# Autodesk Inventor assembly: ABD_Ankle_Version 1.0_MIR
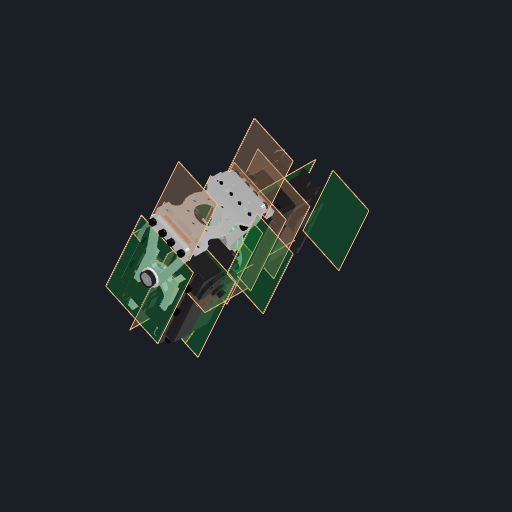
[picture p0: Inventor's stored thumbnail of the model, 512x512]
Saved by Autodesk Inventor 2024 (Build 280153000, 153)
## iProperties
Created: 2024-01-23
Part Number: ABD_Ankle_Version 1.0_MIR
Document SubType Name: Assembly
Designer: ASUS
Mass: 356.311 g
Surface Area: 603.891 cm^2
Volume: 181.117 cm^3
Author: ASUS
## Documents named in this file (21)
- C:\Users\김대겸\Desktop\2024_Robit_Hardware\ROBOCUP_2024_eindhoven\부품\Lower_Body\Anti_Backlash_Disk\ABD_Ankle_Version 1.0_MIR.iam
- C:\Users\김대겸\Desktop\2024_Robit_Hardware\ROBOCUP_2024_eindhoven\부품\ROBOTIS(Inventor 2023 ver.)\다이나믹셀\MX-106T+idle.ipt.iam
- C:\Users\김대겸\Desktop\2024_Robit_Hardware\ROBOCUP_2024_eindhoven\부품\Lower_Body\Anti_Backlash_Disk\Slider_crank_horn.ipt
- C:\Users\김대겸\Desktop\2024_Robit_Hardware\ROBOCUP_2024_eindhoven\부품\Lower_Body\Anti_Backlash_Disk\Leg_joint_slider_frame.ipt
- C:\Users\김대겸\Desktop\2024_Robit_Hardware\ROBOCUP_2024_eindhoven\부품\Lower_Body\Leg\Roll_Fixation_L.ipt
- C:\Users\김대겸\Desktop\2024_Robit_Hardware\ROBOCUP_2024_eindhoven\부품\Lower_Body\Leg\Roll_Fixation_R.ipt
- C:\Users\김대겸\Desktop\2024_Robit_Hardware\ROBOCUP_2024_eindhoven\부품\Lower_Body\Leg\Roll_Fixation_Frame.ipt
- C:\Users\김대겸\Desktop\2024_Robit_Hardware\ROBOCUP_2024_eindhoven\부품\Lower_Body\Leg\Roll_Fixation_Frame_Back.ipt
- C:\Users\김대겸\Desktop\2024_Robit_Hardware\ROBOCUP_2024_eindhoven\부품\Lower_Body\Leg\Roll_Fixation_Frameto64.ipt
- C:\Users\김대겸\Desktop\2024_Robit_Hardware\ROBOCUP_2024_eindhoven\부품\Lower_Body\Leg\106_Slider_Fixation_MIR.ipt
- C:\Users\김대겸\Desktop\2024_Robit_Hardware\ROBOCUP_2024_eindhoven\부품\Lower_Body\Hip joint of the waist\hip joint fix washer.ipt
- C:\Users\김대겸\Desktop\2024_Robit_Hardware\ROBOCUP_2024_eindhoven\부품\Lower_Body\Foot\Ankle_Footbase_Connector.ipt
- C:\Users\김대겸\Desktop\2024_Robit_Hardware\ROBOCUP_2024_eindhoven\부품\Bolt_Washer_Nut\hip_joint_fix_washer_10mm_Set.iam
- C:\Users\김대겸\Desktop\2024_Robit_Hardware\ROBOCUP_2024_eindhoven\부품\Bolt_Washer_Nut\Roll_Fixation_Frame_8mm_Set.iam
- C:\Users\김대겸\Desktop\2024_Robit_Hardware\ROBOCUP_2024_eindhoven\부품\Bolt_Washer_Nut\CSH-ST-M2_5-8_203.ipt
- C:\Users\김대겸\Desktop\2024_Robit_Hardware\ROBOCUP_2024_eindhoven\부품\Bolt_Washer_Nut\ABD_STRUCTURE\Front_Frame_Fixer.iam
- C:\Users\김대겸\Desktop\2024_Robit_Hardware\ROBOCUP_2024_eindhoven\부품\Bolt_Washer_Nut\ABD_STRUCTURE\Crank_Slider_Fixer.iam
- C:\Users\김대겸\Desktop\2024_Robit_Hardware\ROBOCUP_2024_eindhoven\부품\Bolt_Washer_Nut\ABD_STRUCTURE\Rear_Frame_Fixer.iam
- C:\Users\김대겸\Desktop\2024_Robit_Hardware\ROBOCUP_2024_eindhoven\부품\ROBOTIS(Inventor 2023 ver.)\다이나믹셀\MX-64T.ipt
- C:\Users\김대겸\Desktop\2024_Robit_Hardware\ROBOCUP_2024_eindhoven\부품\Bolt_Washer_Nut\ABD_4mm_set.iam
- MX-106T+idle.ipt
## Components (30 placed, 19 different names)
1. MX-106T+idle.ipt:3 [sub-assembly] — 삽입:42, 삽입:43, 삽입:44, 삽입:45, 삽입:74, 메이트:318, 삽입:75, 메이트:319, 삽입:76, 메이트:320, 메이트:321, 삽입:80, 메이트:323
2. Slider_crank_horn:6 — 삽입:87, 메이트:327, 삽입:92, 삽입:95
3. Roll_Fixation_Frame:8 — 메이트:210, 삽입:49, 삽입:50, 삽입:53, 메이트:282, 삽입:90
4. Roll_Fixation_Frame_Back:6 — 메이트:210, 메이트:273, 메이트:274, 삽입:51, 메이트:279, 메이트:280, 메이트:281, 삽입:83, 삽입:86, 메이트:330, 메이트:331, 메이트:332
5. Roll_Fixation_Frameto64:1 — 메이트:273, 메이트:274, 삽입:84, 삽입:85, 메이트:332, 삽입:93, 삽입:94
6. Roll_Fixation_L:6 — 삽입:42, 삽입:43, 삽입:89, 각도:2
7. Roll_Fixation_R:2 — 삽입:44, 삽입:45, 각도:1
8. hip joint fix washer:1 — 삽입:49, 삽입:50, 메이트:280, 메이트:281, 메이트:282, 메이트:324, 삽입:81, 메이트:325
9. hip joint fix washer:2 — 삽입:51, 메이트:279, 삽입:82, 메이트:326
10. Ankle_Footbase_Connector:1 — 삽입:53, 메이트:324, 메이트:330
11. Roll_Fixation_Frame_8mm_Set:4 [sub-assembly] — 삽입:74, 메이트:318
12. Roll_Fixation_Frame_8mm_Set:5 [sub-assembly] — 삽입:75, 메이트:319
13. CSH-ST-M2_5-8_203:9 — 삽입:78
14. CSH-ST-M2_5-8_203:10 — 삽입:79
15. Leg_joint_slider_frame:13 — 삽입:77, 메이트:322, 삽입:78, 삽입:79, 메이트:331, 삽입:91, 메이트:333
16. 106_Slider_Fixation_MIR:2 — 삽입:76, 메이트:320, 메이트:321, 삽입:77, 메이트:322
17. Roll_Fixation_Frame_8mm_Set:6 [sub-assembly] — 삽입:80, 메이트:323
18. hip_joint_fix_washer_10mm_Set:3 [sub-assembly] — 삽입:81, 메이트:325
19. hip_joint_fix_washer_10mm_Set:4 [sub-assembly] — 삽입:82, 메이트:326
20. CSH-ST-M2_5-8_203:11 — 삽입:86
21. CSH-ST-M2_5-8_203:12 — 삽입:83
22. CSH-ST-M2_5-8_203:13 — 삽입:85
23. CSH-ST-M2_5-8_203:14 — 삽입:84
24. MX-64T:2 — 삽입:92, 삽입:93, 삽입:94, 삽입:96, 삽입:97
25. ABD_4mm_set:2 [sub-assembly] — 삽입:87, 메이트:327
26. Front_Frame_Fixer:2 [sub-assembly] — 삽입:89, 삽입:90, 각도:2
27. Rear_Frame_Fixer:2 [sub-assembly] — 삽입:91, 각도:1
28. Crank_Slider_Fixer:1 [sub-assembly] — 삽입:95, 메이트:333
29. CSH-ST-M2_5-8_203:15 — 삽입:96
30. CSH-ST-M2_5-8_203:16 — 삽입:97
## Relationships (54: Insert 31, Mate 21, Angle 2)
- 메이트:210 [Mate]: Roll_Fixation_Frame:8 ↔ Roll_Fixation_Frame_Back:6
- 메이트:273 [Mate]: Roll_Fixation_Frame_Back:6 ↔ Roll_Fixation_Frameto64:1
- 메이트:274 [Mate]: Roll_Fixation_Frame_Back:6 ↔ Roll_Fixation_Frameto64:1
- 삽입:42 [Insert] (0.05 mm): MX-106T+idle.ipt:3 ↔ Roll_Fixation_L:6
- 삽입:43 [Insert] (0.05 mm): MX-106T+idle.ipt:3 ↔ Roll_Fixation_L:6
- 삽입:44 [Insert] (0.05 mm): MX-106T+idle.ipt:3 ↔ Roll_Fixation_R:2
- 삽입:45 [Insert] (0.05 mm): MX-106T+idle.ipt:3 ↔ Roll_Fixation_R:2
- 삽입:49 [Insert]: Roll_Fixation_Frame:8 ↔ hip joint fix washer:1
- 삽입:50 [Insert]: Roll_Fixation_Frame:8 ↔ hip joint fix washer:1
- 삽입:51 [Insert]: Roll_Fixation_Frame_Back:6 ↔ hip joint fix washer:2
- 메이트:279 [Mate]: Roll_Fixation_Frame_Back:6 ↔ hip joint fix washer:2
- 메이트:280 [Mate]: Roll_Fixation_Frame_Back:6 ↔ hip joint fix washer:1
- 메이트:281 [Mate]: Roll_Fixation_Frame_Back:6 ↔ hip joint fix washer:1
- 삽입:53 [Insert]: Roll_Fixation_Frame:8 ↔ Ankle_Footbase_Connector:1
- 메이트:282 [Mate]: Roll_Fixation_Frame:8 ↔ hip joint fix washer:1
- 삽입:74 [Insert]: MX-106T+idle.ipt:3 ↔ Roll_Fixation_Frame_8mm_Set:4
- 메이트:318 [Mate]: MX-106T+idle.ipt:3 ↔ Roll_Fixation_Frame_8mm_Set:4
- 삽입:75 [Insert]: MX-106T+idle.ipt:3 ↔ Roll_Fixation_Frame_8mm_Set:5
- 메이트:319 [Mate]: MX-106T+idle.ipt:3 ↔ Roll_Fixation_Frame_8mm_Set:5
- 삽입:76 [Insert] (0.05 mm): MX-106T+idle.ipt:3 ↔ 106_Slider_Fixation_MIR:2
- 메이트:320 [Mate]: MX-106T+idle.ipt:3 ↔ 106_Slider_Fixation_MIR:2
- 메이트:321 [Mate]: MX-106T+idle.ipt:3 ↔ 106_Slider_Fixation_MIR:2
- 삽입:77 [Insert]: Leg_joint_slider_frame:13 ↔ 106_Slider_Fixation_MIR:2
- 메이트:322 [Mate]: Leg_joint_slider_frame:13 ↔ 106_Slider_Fixation_MIR:2
- 삽입:78 [Insert]: CSH-ST-M2_5-8_203:9 ↔ Leg_joint_slider_frame:13
- 삽입:79 [Insert]: CSH-ST-M2_5-8_203:10 ↔ Leg_joint_slider_frame:13
- 삽입:80 [Insert]: MX-106T+idle.ipt:3 ↔ Roll_Fixation_Frame_8mm_Set:6
- 메이트:323 [Mate]: MX-106T+idle.ipt:3 ↔ Roll_Fixation_Frame_8mm_Set:6
- 메이트:324 [Mate]: hip joint fix washer:1 ↔ Ankle_Footbase_Connector:1
- 삽입:81 [Insert]: hip joint fix washer:1 ↔ hip_joint_fix_washer_10mm_Set:3
- 메이트:325 [Mate]: hip joint fix washer:1 ↔ hip_joint_fix_washer_10mm_Set:3
- 삽입:82 [Insert]: hip joint fix washer:2 ↔ hip_joint_fix_washer_10mm_Set:4
- 메이트:326 [Mate]: hip joint fix washer:2 ↔ hip_joint_fix_washer_10mm_Set:4
- 삽입:83 [Insert]: Roll_Fixation_Frame_Back:6 ↔ CSH-ST-M2_5-8_203:12
- 삽입:84 [Insert]: Roll_Fixation_Frameto64:1 ↔ CSH-ST-M2_5-8_203:14
- 삽입:85 [Insert]: Roll_Fixation_Frameto64:1 ↔ CSH-ST-M2_5-8_203:13
- 삽입:86 [Insert]: Roll_Fixation_Frame_Back:6 ↔ CSH-ST-M2_5-8_203:11
- 삽입:87 [Insert]: Slider_crank_horn:6 ↔ ABD_4mm_set:2
- 메이트:327 [Mate]: Slider_crank_horn:6 ↔ ABD_4mm_set:2
- 삽입:89 [Insert]: Roll_Fixation_L:6 ↔ Front_Frame_Fixer:2
- 삽입:90 [Insert]: Roll_Fixation_Frame:8 ↔ Front_Frame_Fixer:2
- 메이트:330 [Mate]: Roll_Fixation_Frame_Back:6 ↔ Ankle_Footbase_Connector:1
- 메이트:331 [Mate]: Roll_Fixation_Frame_Back:6 ↔ Leg_joint_slider_frame:13
- 삽입:91 [Insert]: Leg_joint_slider_frame:13 ↔ Rear_Frame_Fixer:2
- 메이트:332 [Mate]: Roll_Fixation_Frame_Back:6 ↔ Roll_Fixation_Frameto64:1
- 삽입:92 [Insert]: Slider_crank_horn:6 ↔ MX-64T:2
- 삽입:93 [Insert]: Roll_Fixation_Frameto64:1 ↔ MX-64T:2
- 삽입:94 [Insert]: Roll_Fixation_Frameto64:1 ↔ MX-64T:2
- 삽입:95 [Insert]: Slider_crank_horn:6 ↔ Crank_Slider_Fixer:1
- 메이트:333 [Mate]: Leg_joint_slider_frame:13 ↔ Crank_Slider_Fixer:1
- 삽입:96 [Insert]: MX-64T:2 ↔ CSH-ST-M2_5-8_203:15
- 삽입:97 [Insert]: MX-64T:2 ↔ CSH-ST-M2_5-8_203:16
- 각도:1 [Angle] (0 deg): Roll_Fixation_R:2 ↔ Rear_Frame_Fixer:2
- 각도:2 [Angle] (0 deg): Roll_Fixation_L:6 ↔ Front_Frame_Fixer:2
